# Autodesk Inventor assembly: bunny bot 2013 idea 2
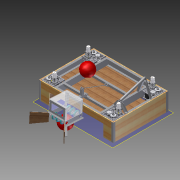
[picture p0: Inventor's stored thumbnail of the model, 180x180]
Saved by Autodesk Inventor 2012 (Build 160160000, 160)
## iProperties
Created: 2013-09-01
Part Number: bunny bot 2013 idea 2
Document SubType Name: Assembly
Designer: Bryce
Author: Bryce
## Documents named in this file (25)
- C:\Users\Bryce\Dropbox\Inventor Design Project Files\Independent Swerves\Inventor 2012\bunny bot 2013 idea 2.iam
- C:\Users\Bryce\Dropbox\Inventor Design Project Files\Independent Swerves\Inventor 2012\FULL SWERVE DRIVE ASSEMBLY!  2!.iam
- C:\Users\Bryce\Dropbox\Inventor Design Project Files\Independent Swerves\Inventor 2012\frame U 1 by 3.ipt
- C:\Users\Bryce\Dropbox\Inventor Design Project Files\Independent Swerves\Inventor 2012\frame U 1 by 3 long.ipt
- C:\Users\Bryce\Dropbox\Inventor Design Project Files\Independent Swerves\Inventor 2012\plywood side pannel.ipt
- C:\Users\Bryce\Dropbox\Inventor Design Project Files\Independent Swerves\Inventor 2012\plywood back pannel 2.ipt
- C:\Users\Bryce\Dropbox\Inventor Design Project Files\Independent Swerves\Inventor 2012\dozer side pannel.ipt
- C:\Users\Bryce\Dropbox\Inventor Design Project Files\Independent Swerves\Inventor 2012\plywood front pannel 2.ipt
- C:\Users\Bryce\Dropbox\Inventor Design Project Files\Independent Swerves\Inventor 2012\dodge ball.ipt
- C:\Users\Bryce\Dropbox\Inventor Design Project Files\Independent Swerves\Inventor 2012\dozer side end mount.ipt
- C:\Users\Bryce\Dropbox\Inventor Design Project Files\Independent Swerves\Inventor 2012\bumper corner bracket.ipt
- C:\Users\Bryce\Dropbox\Inventor Design Project Files\Independent Swerves\Inventor 2012\dozer side mid mount.ipt
- C:\Users\Bryce\Dropbox\Inventor Design Project Files\Independent Swerves\Inventor 2012\frame box 1 by 3.ipt
- C:\Users\Bryce\Dropbox\Inventor Design Project Files\Independent Swerves\Inventor 2012\belly pan.ipt
- C:\Users\Bryce\Dropbox\Inventor Design Project Files\Independent Swerves\Inventor 2012\8 ball frame tube.ipt
- C:\Users\Bryce\Dropbox\Inventor Design Project Files\Independent Swerves\Inventor 2012\8 ball arm pivot.ipt
- C:\Users\Bryce\Dropbox\Inventor Design Project Files\Independent Swerves\Inventor 2012\8 ball top arm tube.ipt
- C:\Users\Bryce\Dropbox\Inventor Design Project Files\Independent Swerves\Inventor 2012\8 ball pnumatic arm tube.ipt
- C:\Users\Bryce\Dropbox\Inventor Design Project Files\Independent Swerves\Inventor 2012\manipulator pnumaitic pivot.ipt
- C:\Users\Bryce\Dropbox\Inventor Design Project Files\Independent Swerves\Inventor 2012\8 ball manipulator piston.ipt
- C:\Users\Bryce\Dropbox\Inventor Design Project Files\Independent Swerves\Inventor 2012\8 ball mechanism 2.iam
- C:\Users\Bryce\Dropbox\Inventor Design Project Files\Independent Swerves\Inventor 2012\bunny throw base 1.ipt
- C:\Users\Bryce\Dropbox\Inventor Design Project Files\Independent Swerves\Inventor 2012\bunny throw base 2.ipt
- C:\Users\Bryce\Dropbox\Inventor Design Project Files\Independent Swerves\Inventor 2012\1' by 1'' dia piston.ipt
- C:\Users\Bryce\Dropbox\Inventor Design Project Files\Independent Swerves\Inventor 2012\bunny throw piston bracket.ipt
## Components (46 placed, 24 different names)
1. FULL SWERVE DRIVE ASSEMBLY!  2!:1 [sub-assembly] — Mate:6, Mate:7, Mate:8
2. FULL SWERVE DRIVE ASSEMBLY!  2!:2 [sub-assembly] — Mate:12, Mate:13, Mate:14
3. FULL SWERVE DRIVE ASSEMBLY!  2!:3 [sub-assembly] — Mate:9, Mate:10, Mate:11
4. FULL SWERVE DRIVE ASSEMBLY!  2!:4 [sub-assembly] — Mate:15, Mate:16, Mate:17, Tangent:1
5. frame U 1 by 3:1 — Mate:1, Mate:2, Flush:1, Mate:5, Mate:14, Mate:15, Mate:35, Flush:8, Flush:26, Flush:27, Flush:51
6. frame U 1 by 3:2 — Mate:3, Mate:4, Flush:2, Flush:3, Mate:6, Mate:7, Mate:9, Mate:10, Mate:34, Flush:6, Flush:25, Flush:28
7. frame U 1 by 3 long:1 — Mate:1, Mate:4, Flush:3, Mate:5, Mate:11, Mate:12, Mate:13, Mate:36, Flush:12, Mate:72, Mate:73, Flush:35, Flush:36, Flush:37, Flush:38
8. frame U 1 by 3 long:2 — Mate:2, Mate:3, Flush:1, Flush:2, Mate:8, Mate:16, Mate:17, Flush:7, Flush:9, Flush:13, Mate:46
9. plywood side pannel:1 — Mate:34, Flush:6, Flush:7, Mate:43, Flush:14, Mate:60, Mate:66, Flush:24, Mate:70, Mate:71, Mate:75
10. plywood side pannel:2 — Mate:35, Flush:8, Flush:9, Mate:37, Mate:45, Mate:62, Mate:67, Flush:23, Mate:68, Mate:69
11. plywood back pannel 2:1 — Mate:36, Flush:12, Mate:37, Mate:38, Mate:39, Angle:1, Mate:48, Mate:49, Mate:50, Mate:51, Flush:15, Flush:16, Flush:17, Flush:18, Flush:21, Flush:22, Flush:30, Flush:31, Mate:74
12. dozer side pannel:1 — Mate:38, Mate:43, Mate:53, Mate:55, Mate:56, Flush:29, Flush:30, Flush:32
13. dozer side pannel:2 — Mate:39, Mate:45, Mate:52, Mate:54, Mate:57, Flush:31, Flush:33, Flush:34
14. plywood front pannel 2:2 — Flush:13, Mate:46, Flush:14, Mate:58, Mate:59, Flush:19, Flush:20, Mate:61, Mate:63, Mate:64, Mate:65
15. dodge ball:1 — Tangent:2
16. dozer side end mount:1 — Mate:50, Mate:55, Flush:17
17. dozer side end mount:2 — Mate:48, Mate:53, Flush:18
18. dozer side end mount:3 — Mate:49, Mate:52, Flush:16
19. dozer side end mount:4 — Mate:51, Mate:54, Flush:15
20. dozer side end mount:5 — Mate:56, Mate:59, Flush:19
21. dozer side end mount:6 — Mate:57, Mate:58, Flush:20
22. bumper corner bracket:1 — Mate:62, Mate:67, Flush:22
23. bumper corner bracket:2 — Mate:60, Mate:66, Flush:21
24. bumper corner bracket:3 — Mate:61, Mate:65, Flush:24, Flush:41, Flush:42
25. bumper corner bracket:4 — Mate:63, Mate:64, Flush:23, Flush:44
26. dozer side mid mount:1 — Mate:71, Flush:25, Flush:29
27. dozer side mid mount:2 — Mate:70, Flush:28, Flush:32
28. dozer side mid mount:3 — Mate:68, Flush:27, Flush:34
29. dozer side mid mount:4 — Mate:69, Flush:26, Flush:33
30. frame box 1 by 3:1 — Mate:73, Flush:37, Flush:38, Mate:76, Mate:77, Mate:78, Flush:39, Flush:40
31. frame box 1 by 3:2 — Mate:72, Flush:35, Flush:36, Flush:47, Mate:92, Flush:48, Mate:93
32. belly pan:1 — Mate:74, Mate:75, Mate:76
33. 8 ball frame tube:1 — Mate:77, Flush:39, Flush:41, Mate:79, Flush:43
34. 8 ball frame tube:2 — Mate:78, Flush:40, Flush:42, Mate:84, Flush:46
35. 8 ball arm pivot:1 — Mate:79, Flush:43, Flush:44, Mate:80, Mate:81
36. 8 ball top arm tube:1 — Mate:80, Mate:81, Mate:82, Flush:45, Mate:83, Mate:85, Mate:89, Mate:90, Mate:91
37. 8 ball pnumatic arm tube:1 — Mate:82, Flush:45, Mate:83, Mate:86
38. manipulator pnumaitic pivot:1 — Mate:84, Mate:85, Flush:46, Mate:87, Mate:88
39. 8 ball manipulator piston:1 — Mate:86, Mate:87, Mate:88
40. 8 ball mechanism 2:1 [sub-assembly] — Mate:89, Mate:90, Mate:91
41. dodge ball:2
42. bunny throw base 1:1 — Flush:47, Mate:92, Mate:94, Flush:49, Mate:95, Mate:96, Flush:51
43. bunny throw base 2:1 — Flush:48, Mate:93, Mate:94, Flush:50, Mate:99, Mate:100
44. 1' by 1'' dia piston:1 — Mate:97, Mate:98, Mate:101
45. manipulator pnumaitic pivot:2 — Flush:49, Mate:95, Mate:96, Mate:97, Mate:98
46. bunny throw piston bracket:1 — Flush:50, Mate:99, Mate:100, Mate:101
## Relationships (130: Mate 80, Flush 47, Tangent 2, Angle 1)
- Mate:1: frame U 1 by 3:1 ↔ frame U 1 by 3 long:1
- Mate:2: frame U 1 by 3:1 ↔ frame U 1 by 3 long:2
- Mate:3: frame U 1 by 3:2 ↔ frame U 1 by 3 long:2
- Mate:4: frame U 1 by 3:2 ↔ frame U 1 by 3 long:1
- Flush:1: frame U 1 by 3:1 ↔ frame U 1 by 3 long:2
- Flush:2: frame U 1 by 3:2 ↔ frame U 1 by 3 long:2
- Flush:3: frame U 1 by 3:2 ↔ frame U 1 by 3 long:1
- Mate:5: frame U 1 by 3:1 ↔ frame U 1 by 3 long:1
- Mate:6: FULL SWERVE DRIVE ASSEMBLY!  2!:1 ↔ frame U 1 by 3:2
- Mate:7: FULL SWERVE DRIVE ASSEMBLY!  2!:1 ↔ frame U 1 by 3:2
- Mate:8: FULL SWERVE DRIVE ASSEMBLY!  2!:1 ↔ frame U 1 by 3 long:2
- Mate:9: FULL SWERVE DRIVE ASSEMBLY!  2!:3 ↔ frame U 1 by 3:2
- Mate:10: FULL SWERVE DRIVE ASSEMBLY!  2!:3 ↔ frame U 1 by 3:2
- Mate:11: FULL SWERVE DRIVE ASSEMBLY!  2!:3 ↔ frame U 1 by 3 long:1
- Mate:12: FULL SWERVE DRIVE ASSEMBLY!  2!:2 ↔ frame U 1 by 3 long:1
- Mate:13: FULL SWERVE DRIVE ASSEMBLY!  2!:2 ↔ frame U 1 by 3 long:1
- Mate:14: FULL SWERVE DRIVE ASSEMBLY!  2!:2 ↔ frame U 1 by 3:1
- Mate:15: FULL SWERVE DRIVE ASSEMBLY!  2!:4 ↔ frame U 1 by 3:1
- Mate:16: FULL SWERVE DRIVE ASSEMBLY!  2!:4 ↔ frame U 1 by 3 long:2
- Mate:17: FULL SWERVE DRIVE ASSEMBLY!  2!:4 ↔ frame U 1 by 3 long:2
- Mate:34: frame U 1 by 3:2 ↔ plywood side pannel:1
- Flush:6: frame U 1 by 3:2 ↔ plywood side pannel:1
- Flush:7: frame U 1 by 3 long:2 ↔ plywood side pannel:1
- Mate:35: frame U 1 by 3:1 ↔ plywood side pannel:2
- Flush:8: frame U 1 by 3:1 ↔ plywood side pannel:2
- Flush:9: frame U 1 by 3 long:2 ↔ plywood side pannel:2
- Mate:36: frame U 1 by 3 long:1 ↔ plywood back pannel 2:1
- Flush:12: frame U 1 by 3 long:1 ↔ plywood back pannel 2:1
- Mate:37: plywood side pannel:2 ↔ plywood back pannel 2:1
- Mate:38: plywood back pannel 2:1 ↔ dozer side pannel:1
- Mate:39: plywood back pannel 2:1 ↔ dozer side pannel:2
- Mate:43 (114.3 mm): plywood side pannel:1 ↔ dozer side pannel:1
- Mate:45 (114.3 mm): plywood side pannel:2 ↔ dozer side pannel:2
- Flush:13: frame U 1 by 3 long:2 ↔ plywood front pannel 2:2
- Mate:46: frame U 1 by 3 long:2 ↔ plywood front pannel 2:2
- Flush:14: plywood side pannel:1 ↔ plywood front pannel 2:2
- Angle:1 (0 deg): plywood back pannel 2:1
- Tangent:1: FULL SWERVE DRIVE ASSEMBLY!  2!:4
- Tangent:2: dodge ball:1
- Mate:48: plywood back pannel 2:1 ↔ dozer side end mount:2
- Mate:49: plywood back pannel 2:1 ↔ dozer side end mount:3
- Mate:50: plywood back pannel 2:1 ↔ dozer side end mount:1
- Mate:51: plywood back pannel 2:1 ↔ dozer side end mount:4
- Mate:52: dozer side pannel:2 ↔ dozer side end mount:3
- Mate:53: dozer side pannel:1 ↔ dozer side end mount:2
- Mate:54: dozer side pannel:2 ↔ dozer side end mount:4
- Flush:15: plywood back pannel 2:1 ↔ dozer side end mount:4
- Flush:16: plywood back pannel 2:1 ↔ dozer side end mount:3
- Mate:55: dozer side pannel:1 ↔ dozer side end mount:1
- Flush:17: plywood back pannel 2:1 ↔ dozer side end mount:1
- Flush:18: plywood back pannel 2:1 ↔ dozer side end mount:2
- Mate:56: dozer side pannel:1 ↔ dozer side end mount:5
- Mate:57: dozer side pannel:2 ↔ dozer side end mount:6
- Mate:58: plywood front pannel 2:2 ↔ dozer side end mount:6
- Mate:59: plywood front pannel 2:2 ↔ dozer side end mount:5
- Flush:19: plywood front pannel 2:2 ↔ dozer side end mount:5
- Flush:20: plywood front pannel 2:2 ↔ dozer side end mount:6
- Mate:60: plywood side pannel:1 ↔ bumper corner bracket:2
- Mate:61: plywood front pannel 2:2 ↔ bumper corner bracket:3
- Mate:62: plywood side pannel:2 ↔ bumper corner bracket:1
- Mate:63: plywood front pannel 2:2 ↔ bumper corner bracket:4
- Mate:64: plywood front pannel 2:2 ↔ bumper corner bracket:4
- Mate:65: plywood front pannel 2:2 ↔ bumper corner bracket:3
- Mate:66: plywood side pannel:1 ↔ bumper corner bracket:2
- Mate:67: plywood side pannel:2 ↔ bumper corner bracket:1
- Flush:21: plywood back pannel 2:1 ↔ bumper corner bracket:2
- Flush:22: plywood back pannel 2:1 ↔ bumper corner bracket:1
- Flush:23: plywood side pannel:2 ↔ bumper corner bracket:4
- Flush:24: plywood side pannel:1 ↔ bumper corner bracket:3
- Mate:68: plywood side pannel:2 ↔ dozer side mid mount:3
- Mate:69: plywood side pannel:2 ↔ dozer side mid mount:4
- Mate:70: plywood side pannel:1 ↔ dozer side mid mount:2
- Mate:71: plywood side pannel:1 ↔ dozer side mid mount:1
- Flush:25: frame U 1 by 3:2 ↔ dozer side mid mount:1
- Flush:26: frame U 1 by 3:1 ↔ dozer side mid mount:4
- Flush:27: frame U 1 by 3:1 ↔ dozer side mid mount:3
- Flush:28: frame U 1 by 3:2 ↔ dozer side mid mount:2
- Flush:29: dozer side pannel:1 ↔ dozer side mid mount:1
- Flush:30: plywood back pannel 2:1 ↔ dozer side pannel:1
- Flush:31: plywood back pannel 2:1 ↔ dozer side pannel:2
- Flush:32: dozer side pannel:1 ↔ dozer side mid mount:2
- Flush:33: dozer side pannel:2 ↔ dozer side mid mount:4
- Flush:34: dozer side pannel:2 ↔ dozer side mid mount:3
- Mate:72: frame U 1 by 3 long:1 ↔ frame box 1 by 3:2
- Mate:73: frame U 1 by 3 long:1 ↔ frame box 1 by 3:1
- Flush:35: frame U 1 by 3 long:1 ↔ frame box 1 by 3:2
- Flush:36: frame U 1 by 3 long:1 ↔ frame box 1 by 3:2
- Flush:37: frame U 1 by 3 long:1 ↔ frame box 1 by 3:1
- Flush:38: frame U 1 by 3 long:1 ↔ frame box 1 by 3:1
- Mate:74: plywood back pannel 2:1 ↔ belly pan:1
- Mate:75: plywood side pannel:1 ↔ belly pan:1
- Mate:76: frame box 1 by 3:1 ↔ belly pan:1
- Mate:77: frame box 1 by 3:1 ↔ 8 ball frame tube:1
- Mate:78: frame box 1 by 3:1 ↔ 8 ball frame tube:2
- Flush:39: frame box 1 by 3:1 ↔ 8 ball frame tube:1
- Flush:40: frame box 1 by 3:1 ↔ 8 ball frame tube:2
- Flush:41 (114.3 mm): bumper corner bracket:3 ↔ 8 ball frame tube:1
- Flush:42 (400.05 mm): bumper corner bracket:3 ↔ 8 ball frame tube:2
- Mate:79: 8 ball frame tube:1 ↔ 8 ball arm pivot:1
- Flush:43: 8 ball frame tube:1 ↔ 8 ball arm pivot:1
- Flush:44 (441.325 mm): bumper corner bracket:4 ↔ 8 ball arm pivot:1
- Mate:80: 8 ball arm pivot:1 ↔ 8 ball top arm tube:1
- Mate:81 (3.175 mm): 8 ball arm pivot:1 ↔ 8 ball top arm tube:1
- Mate:82: 8 ball top arm tube:1 ↔ 8 ball pnumatic arm tube:1
- Flush:45: 8 ball top arm tube:1 ↔ 8 ball pnumatic arm tube:1
- Mate:83 (40.64 mm): 8 ball top arm tube:1 ↔ 8 ball pnumatic arm tube:1
- Mate:84: 8 ball frame tube:2 ↔ manipulator pnumaitic pivot:1
- Mate:85: 8 ball top arm tube:1 ↔ manipulator pnumaitic pivot:1
- Flush:46: 8 ball frame tube:2 ↔ manipulator pnumaitic pivot:1
- Mate:86: 8 ball pnumatic arm tube:1 ↔ 8 ball manipulator piston:1
- Mate:87: manipulator pnumaitic pivot:1 ↔ 8 ball manipulator piston:1
- Mate:88 (6.35 mm): manipulator pnumaitic pivot:1 ↔ 8 ball manipulator piston:1
- Mate:89: 8 ball top arm tube:1 ↔ 8 ball mechanism 2:1
- Mate:90: 8 ball top arm tube:1 ↔ 8 ball mechanism 2:1
- Mate:91: 8 ball top arm tube:1 ↔ 8 ball mechanism 2:1
- Flush:47: frame box 1 by 3:2 ↔ bunny throw base 1:1
- Mate:92: frame box 1 by 3:2 ↔ bunny throw base 1:1
- Flush:48: frame box 1 by 3:2 ↔ bunny throw base 2:1
- Mate:93: frame box 1 by 3:2 ↔ bunny throw base 2:1
- Mate:94 (298.45 mm): bunny throw base 1:1 ↔ bunny throw base 2:1
- Flush:49: bunny throw base 1:1 ↔ manipulator pnumaitic pivot:2
- Mate:95: bunny throw base 1:1 ↔ manipulator pnumaitic pivot:2
- Mate:96 (-3.175 mm): bunny throw base 1:1 ↔ manipulator pnumaitic pivot:2
- Mate:97: 1' by 1'' dia piston:1 ↔ manipulator pnumaitic pivot:2
- Mate:98 (6.35 mm): 1' by 1'' dia piston:1 ↔ manipulator pnumaitic pivot:2
- Flush:50: bunny throw base 2:1 ↔ bunny throw piston bracket:1
- Mate:99: bunny throw base 2:1 ↔ bunny throw piston bracket:1
- Mate:100 (-1.5875 mm): bunny throw base 2:1 ↔ bunny throw piston bracket:1
- Mate:101: 1' by 1'' dia piston:1 ↔ bunny throw piston bracket:1
- Flush:51: frame U 1 by 3:1 ↔ bunny throw base 1:1
